(part 1 of 3)
# Autodesk Inventor assembly: COMPONENTS
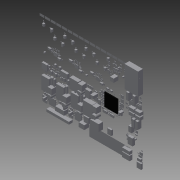
[picture p0: Inventor's stored thumbnail of the model, 180x180]
Saved by Autodesk Inventor 2016 (Build 200138000, 138)
## iProperties
Created: 2016-03-07
Part Number: COMPONENTS
Document SubType Name: Assembly
Designer: rtreacy
Author: rtreacy
## Documents named in this file (794)
- C:\Users\Dave\Desktop\hera-cad\SNAP\components\COMPONENTS.iam
- C:\Users\Dave\Desktop\hera-cad\SNAP\components\INDC1005X55L_L30.ipt
- C:\Users\Dave\Desktop\hera-cad\SNAP\components\INDC1005X55L_L31.ipt
- C:\Users\Dave\Desktop\hera-cad\SNAP\NRAO-LOGO_NOREFDES.ipt
- C:\Users\Dave\Desktop\hera-cad\SNAP\components\MOLEX_SD-74754-0220_M23.ipt
- C:\Users\Dave\Desktop\hera-cad\SNAP\SHDRRA14W55P200_7X2_1665X100-1_J11.ipt
- C:\Users\Dave\Desktop\hera-cad\SNAP\SHDRV14W55P200_7X2_1665X630H-1_J3.ipt
- C:\Users\Dave\Desktop\hera-cad\SNAP\components\TE_CONN_6367550-5_P3.ipt
- C:\Users\Dave\Desktop\hera-cad\SNAP\TO170P1430X470-6N-ALT1_U18.ipt
- C:\Users\Dave\Desktop\hera-cad\SNAP\components\SMA_END_LAUNCH_SMATP1.ipt
- C:\Users\Dave\Desktop\hera-cad\SNAP\components\SMA_END_LAUNCH_SMATP2.ipt
- C:\Users\Dave\Desktop\hera-cad\SNAP\components\SMA_END_LAUNCH_SMATP3.ipt
- C:\Users\Dave\Desktop\hera-cad\SNAP\components\SMA_END_LAUNCH_SMATP4.ipt
- C:\Users\Dave\Desktop\hera-cad\SNAP\components\SMA_END_LAUNCH_SMATP5.ipt
- C:\Users\Dave\Desktop\hera-cad\SNAP\components\SMA_END_LAUNCH_SMATP6.ipt
- C:\Users\Dave\Desktop\hera-cad\SNAP\components\SMA_END_LAUNCH_SMATP7.ipt
- C:\Users\Dave\Desktop\hera-cad\SNAP\components\SMA_END_LAUNCH_SMATP8.ipt
- C:\Users\Dave\Desktop\hera-cad\SNAP\components\SMA_END_LAUNCH_SMATP9.ipt
- C:\Users\Dave\Desktop\hera-cad\SNAP\components\SMA_END_LAUNCH_SMATP10.ipt
- C:\Users\Dave\Desktop\hera-cad\SNAP\components\SMA_END_LAUNCH_SMATP11.ipt
- C:\Users\Dave\Desktop\hera-cad\SNAP\components\SMA_END_LAUNCH_SMATP12.ipt
- C:\Users\Dave\Desktop\hera-cad\SNAP\components\SMA_END_LAUNCH_SMATP13.ipt
- C:\Users\Dave\Desktop\hera-cad\SNAP\components\SMA_END_LAUNCH_SMATP14.ipt
- C:\Users\Dave\Desktop\hera-cad\SNAP\components\SMA_END_LAUNCH_SMATP15.ipt
- C:\Users\Dave\Desktop\hera-cad\SNAP\components\SMA_END_LAUNCH_SMATP16.ipt
- C:\Users\Dave\Desktop\hera-cad\SNAP\components\HDRV254W64P254R1L508T254H838_JP3.ipt
- C:\Users\Dave\Desktop\hera-cad\SNAP\components\HDRV254W64P254R1L508T254H838_JP2.ipt
- C:\Users\Dave\Desktop\hera-cad\SNAP\components\HDRV254W64P254R1L508T254H838_JP1.ipt
- C:\Users\Dave\Desktop\hera-cad\SNAP\components\HDRV254W64P254R1L508T254H838_JP4.ipt
- C:\Users\Dave\Desktop\hera-cad\SNAP\components\HDRV6X2_J9.ipt
- C:\Users\Dave\Desktop\hera-cad\SNAP\components\HDRV6X2_J7.ipt
- C:\Users\Dave\Desktop\hera-cad\SNAP\components\HDRV6X2_J5.ipt
- C:\Users\Dave\Desktop\hera-cad\SNAP\components\HDRV6X2_J6.ipt
- C:\Users\Dave\Desktop\hera-cad\SNAP\components\HDRV2X20_PI2.ipt
- C:\Users\Dave\Desktop\hera-cad\SNAP\components\CAPPRD350W60D820H1170P_C259.ipt
- C:\Users\Dave\Desktop\hera-cad\SNAP\components\CAPPRD350W60D820H1170P_C250.ipt
- C:\Users\Dave\Desktop\hera-cad\SNAP\components\CAPPRD350W60D820H1170P_C241.ipt
- C:\Users\Dave\Desktop\hera-cad\SNAP\components\CAPPRD350W60D820H1170P_C234.ipt
- C:\Users\Dave\Desktop\hera-cad\SNAP\components\CAPPRD350W60D820H1170P_C227.ipt
- C:\Users\Dave\Desktop\hera-cad\SNAP\components\QFN50P500X500X100-28N_U29.ipt
- C:\Users\Dave\Desktop\hera-cad\SNAP\components\FID100X125_NOREFDES.ipt
- C:\Users\Dave\Desktop\hera-cad\SNAP\components\DIOAD1365W102L865D350B_D4.ipt
- C:\Users\Dave\Desktop\hera-cad\SNAP\components\DIOAD1365W102L865D350B_D5.ipt
- C:\Users\Dave\Desktop\hera-cad\SNAP\components\DIOAD1365W102L865D350B_D6.ipt
- C:\Users\Dave\Desktop\hera-cad\SNAP\components\DIOAD1365W102L865D350B_D7.ipt
- C:\Users\Dave\Desktop\hera-cad\SNAP\components\DIOAD1365W102L865D350B_D8.ipt
- C:\Users\Dave\Desktop\hera-cad\SNAP\BGA676C100P26X26_2700X2700X260_U25.ipt
- C:\Users\Dave\Desktop\hera-cad\SNAP\components\EMERSON_RFCONN_SMA-V_TP2.ipt
- C:\Users\Dave\Desktop\hera-cad\SNAP\components\FIL_BNX01X_U24.ipt
- C:\Users\Dave\Desktop\hera-cad\SNAP\components\MOLEX_744410010_P2.ipt
- C:\Users\Dave\Desktop\hera-cad\SNAP\components\MOLEX_744410010_P1.ipt
- C:\Users\Dave\Desktop\hera-cad\SNAP\components\SOT89_Q5.ipt
- C:\Users\Dave\Desktop\hera-cad\SNAP\components\SOT89_Q6.ipt
- C:\Users\Dave\Desktop\hera-cad\SNAP\components\QFN80P1000X1000X440-42T320X130X2N-ALT1_U20.ipt
- C:\Users\Dave\Desktop\hera-cad\SNAP\components\HDR_1X2_LOCK_MOLEX_J61.ipt
- C:\Users\Dave\Desktop\hera-cad\SNAP\components\DIOMELF3514_D14.ipt
- C:\Users\Dave\Desktop\hera-cad\SNAP\components\SOT230P700X180-4L050N_Q17.ipt
- C:\Users\Dave\Desktop\hera-cad\SNAP\components\QFP50P1400X1400X100-80N_U40.ipt
- C:\Users\Dave\Desktop\hera-cad\SNAP\components\QFP50P1400X1400X100-80N_U42.ipt
- C:\Users\Dave\Desktop\hera-cad\SNAP\components\QFN50P700X700X100-49T540X540L_U7.ipt
- C:\Users\Dave\Desktop\hera-cad\SNAP\components\QFN50P700X700X100-49T540X540L_U2.ipt
- C:\Users\Dave\Desktop\hera-cad\SNAP\components\QFN50P700X700X100-49T540X540L_U12.ipt
- C:\Users\Dave\Desktop\hera-cad\SNAP\components\QFN50P500X500X100-33T320X320L_U21.ipt
- C:\Users\Dave\Desktop\hera-cad\SNAP\components\QFN50P500X500X100-33T380X380L_U23.ipt
- C:\Users\Dave\Desktop\hera-cad\SNAP\components\QFN50P400X400X100-25T280X280L_U22.ipt
- C:\Users\Dave\Desktop\hera-cad\SNAP\components\DCDC-CONV_PTD08D210W-22N_U38.ipt
- C:\Users\Dave\Desktop\hera-cad\SNAP\components\DCDC-CONV_PTD08D210W-22N_U36.ipt
- C:\Users\Dave\Desktop\hera-cad\SNAP\components\DCDC-CONV_PTD08D210W-22N_U37.ipt
- C:\Users\Dave\Desktop\hera-cad\SNAP\components\QFN50P300X300X100-17T178X178L_U17.ipt
- C:\Users\Dave\Desktop\hera-cad\SNAP\components\QFN50P300X300X100-17T178X178L_U16.ipt
- C:\Users\Dave\Desktop\hera-cad\SNAP\components\SOP65P640X120-16N_U41.ipt
- C:\Users\Dave\Desktop\hera-cad\SNAP\components\SOP65P640X120-16N_U39.ipt
- C:\Users\Dave\Desktop\hera-cad\SNAP\components\QFN40P260X180X55-16L_U28.ipt
- C:\Users\Dave\Desktop\hera-cad\SNAP\components\QFN40P260X180X55-16L_U46.ipt
- C:\Users\Dave\Desktop\hera-cad\SNAP\components\QFN40P260X180X55-16L_U47.ipt
- C:\Users\Dave\Desktop\hera-cad\SNAP\components\DCDC-CONV_PTD08A020WAD-12N_U35.ipt
- C:\Users\Dave\Desktop\hera-cad\SNAP\components\DCDC-CONV_PTD08A010WAD-12N_U34.ipt
- C:\Users\Dave\Desktop\hera-cad\SNAP\components\HDRV1016W64P254R2L2032T905H900_J1.ipt
- C:\Users\Dave\Desktop\hera-cad\SNAP\components\SW_SDA05H1SBD_S2.ipt
- C:\Users\Dave\Desktop\hera-cad\SNAP\components\SW_SDA05H1SBD_S1.ipt
- C:\Users\Dave\Desktop\hera-cad\SNAP\components\MOLEX_548190589_J4.ipt
- C:\Users\Dave\Desktop\hera-cad\SNAP\components\SOP50P310X90-8N_U44.ipt
- C:\Users\Dave\Desktop\hera-cad\SNAP\components\SOP50P310X90-8N_U45.ipt
- C:\Users\Dave\Desktop\hera-cad\SNAP\components\OSC254P700X500X90-7T147X230N_U32.ipt
- C:\Users\Dave\Desktop\hera-cad\SNAP\components\MOLEX_39301060_J2.ipt
- C:\Users\Dave\Desktop\hera-cad\SNAP\components\SOT95P280X145-6N_U26.ipt
- C:\Users\Dave\Desktop\hera-cad\SNAP\components\OSC254P700X500X90-6N_U48.ipt
- C:\Users\Dave\Desktop\hera-cad\SNAP\components\OSC254P700X500X90-6N_U33.ipt
- C:\Users\Dave\Desktop\hera-cad\SNAP\components\XFMR_TC1-1-13MG2_T11.ipt
- C:\Users\Dave\Desktop\hera-cad\SNAP\components\XFMR_TC1-1-13MG2_T10.ipt
- C:\Users\Dave\Desktop\hera-cad\SNAP\components\XFMR_TC1-1-13MG2_T4.ipt
- C:\Users\Dave\Desktop\hera-cad\SNAP\components\XFMR_TC1-1-13MG2_T6.ipt
- C:\Users\Dave\Desktop\hera-cad\SNAP\components\XFMR_TC1-1-13MG2_T12.ipt
- C:\Users\Dave\Desktop\hera-cad\SNAP\components\XFMR_TC1-1-13MG2_T5.ipt
- C:\Users\Dave\Desktop\hera-cad\SNAP\components\XFMR_TC1-1-13MG2_T3.ipt
- C:\Users\Dave\Desktop\hera-cad\SNAP\components\XFMR_TC1-1-13MG2_T8.ipt
- C:\Users\Dave\Desktop\hera-cad\SNAP\components\XFMR_TC1-1-13MG2_T9.ipt
- C:\Users\Dave\Desktop\hera-cad\SNAP\components\XFMR_TC1-1-13MG2_T13.ipt
- C:\Users\Dave\Desktop\hera-cad\SNAP\components\XFMR_TC1-1-13MG2_T2.ipt
- C:\Users\Dave\Desktop\hera-cad\SNAP\components\XFMR_TC1-1-13MG2_T7.ipt
- C:\Users\Dave\Desktop\hera-cad\SNAP\components\XFMR_TC1-1-13MG2_T1.ipt
- C:\Users\Dave\Desktop\hera-cad\SNAP\components\SOT95P280X145-5N_U30.ipt
- C:\Users\Dave\Desktop\hera-cad\SNAP\components\SOT95P280X145-5N_U19.ipt
- C:\Users\Dave\Desktop\hera-cad\SNAP\components\SOT143R_X1.ipt
- C:\Users\Dave\Desktop\hera-cad\SNAP\components\RESCAF65P100X100X45-4N_U10.ipt
- C:\Users\Dave\Desktop\hera-cad\SNAP\components\RESCAF65P100X100X45-4N_U1.ipt
- C:\Users\Dave\Desktop\hera-cad\SNAP\components\RESCAF65P100X100X45-4N_U11.ipt
- C:\Users\Dave\Desktop\hera-cad\SNAP\components\RESCAF65P100X100X45-4N_U13.ipt
- C:\Users\Dave\Desktop\hera-cad\SNAP\components\RESCAF65P100X100X45-4N_U14.ipt
- C:\Users\Dave\Desktop\hera-cad\SNAP\components\RESCAF65P100X100X45-4N_U15.ipt
- C:\Users\Dave\Desktop\hera-cad\SNAP\components\RESCAF65P100X100X45-4N_U3.ipt
- C:\Users\Dave\Desktop\hera-cad\SNAP\components\RESCAF65P100X100X45-4N_U4.ipt
- C:\Users\Dave\Desktop\hera-cad\SNAP\components\RESCAF65P100X100X45-4N_U5.ipt
- C:\Users\Dave\Desktop\hera-cad\SNAP\components\RESCAF65P100X100X45-4N_U6.ipt
- C:\Users\Dave\Desktop\hera-cad\SNAP\components\RESCAF65P100X100X45-4N_U8.ipt
- C:\Users\Dave\Desktop\hera-cad\SNAP\components\RESCAF65P100X100X45-4N_U9.ipt
- C:\Users\Dave\Desktop\hera-cad\SNAP\components\SW_TL3301EF100QG_SW5.ipt
- C:\Users\Dave\Desktop\hera-cad\SNAP\components\SW_TL3301EF100QG_SW4.ipt
- C:\Users\Dave\Desktop\hera-cad\SNAP\components\SW_TL3301EF100QG_SW3.ipt
- C:\Users\Dave\Desktop\hera-cad\SNAP\components\SW_TL3301EF100QG_SW2.ipt
- C:\Users\Dave\Desktop\hera-cad\SNAP\components\SW_TL3301EF100QG_SW1.ipt
- C:\Users\Dave\Desktop\hera-cad\SNAP\components\SOT192P237X112-4L20N_D3.ipt
- C:\Users\Dave\Desktop\hera-cad\SNAP\components\SOT95P237X100-4_Q1.ipt
- C:\Users\Dave\Desktop\hera-cad\SNAP\components\SOT95P237X100-4_Q4.ipt
- C:\Users\Dave\Desktop\hera-cad\SNAP\components\SOT95P237X100-4_Q3.ipt
- C:\Users\Dave\Desktop\hera-cad\SNAP\components\SOT95P237X100-4_Q2.ipt
- C:\Users\Dave\Desktop\hera-cad\SNAP\components\SOT95P237X100-4_Q8.ipt
- C:\Users\Dave\Desktop\hera-cad\SNAP\components\SOT95P237X100-4_Q7.ipt
- C:\Users\Dave\Desktop\hera-cad\SNAP\components\SOT95P240X110-3L16N_U31.ipt
- C:\Users\Dave\Desktop\hera-cad\SNAP\components\SOT95P240X110-3L16N_D1.ipt
- C:\Users\Dave\Desktop\hera-cad\SNAP\components\SOT95P240X110-3L16N_D2.ipt
- C:\Users\Dave\Desktop\hera-cad\SNAP\components\CAPC1005X50L_C604.ipt
- C:\Users\Dave\Desktop\hera-cad\SNAP\components\CAPC1005X50L_C603.ipt
- C:\Users\Dave\Desktop\hera-cad\SNAP\components\CAPC1005X50L_C591.ipt
- C:\Users\Dave\Desktop\hera-cad\SNAP\components\CAPC1005X50L_C592.ipt
- C:\Users\Dave\Desktop\hera-cad\SNAP\components\CAPC1005X50L_C593.ipt
- C:\Users\Dave\Desktop\hera-cad\SNAP\components\CAPC1005X50L_C46.ipt
- C:\Users\Dave\Desktop\hera-cad\SNAP\components\CAPC1005X50L_C51.ipt
- C:\Users\Dave\Desktop\hera-cad\SNAP\components\CAPC1005X50L_C57.ipt
- C:\Users\Dave\Desktop\hera-cad\SNAP\components\CAPC1005X50L_C7.ipt
- C:\Users\Dave\Desktop\hera-cad\SNAP\components\CAPC1005X50L_C82.ipt
- C:\Users\Dave\Desktop\hera-cad\SNAP\components\CAPC1005X50L_C43.ipt
- C:\Users\Dave\Desktop\hera-cad\SNAP\components\CAPC1005X50L_C96.ipt
- C:\Users\Dave\Desktop\hera-cad\SNAP\components\CAPC1005X50L_C85.ipt
- C:\Users\Dave\Desktop\hera-cad\SNAP\components\CAPC1005X50L_C90.ipt
- C:\Users\Dave\Desktop\hera-cad\SNAP\components\CAPC1005X50L_C13.ipt
- C:\Users\Dave\Desktop\hera-cad\SNAP\components\CAPC1005X50L_C4.ipt
- C:\Users\Dave\Desktop\hera-cad\SNAP\components\CAPC1005X50L_C47.ipt
- C:\Users\Dave\Desktop\hera-cad\SNAP\components\CAPC1005X50L_C5.ipt
- C:\Users\Dave\Desktop\hera-cad\SNAP\components\CAPC1005X50L_C52.ipt
- C:\Users\Dave\Desktop\hera-cad\SNAP\components\CAPC1005X50L_C58.ipt
- C:\Users\Dave\Desktop\hera-cad\SNAP\components\CAPC1005X50L_C8.ipt
- C:\Users\Dave\Desktop\hera-cad\SNAP\components\CAPC1005X50L_C83.ipt
- C:\Users\Dave\Desktop\hera-cad\SNAP\components\CAPC1005X50L_C86.ipt
- C:\Users\Dave\Desktop\hera-cad\SNAP\components\CAPC1005X50L_C91.ipt
- C:\Users\Dave\Desktop\hera-cad\SNAP\components\CAPC1005X50L_C97.ipt
- C:\Users\Dave\Desktop\hera-cad\SNAP\components\CAPC1005X50L_C19.ipt
- C:\Users\Dave\Desktop\hera-cad\SNAP\components\CAPC1005X50L_C14.ipt
- C:\Users\Dave\Desktop\hera-cad\SNAP\components\CAPC1005X50L_C17.ipt
- C:\Users\Dave\Desktop\hera-cad\SNAP\components\CAPC1005X50L_C2.ipt
- C:\Users\Dave\Desktop\hera-cad\SNAP\components\CAPC1005X50L_C41.ipt
- C:\Users\Dave\Desktop\hera-cad\SNAP\components\CAPC1005X50L_C44.ipt
- C:\Users\Dave\Desktop\hera-cad\SNAP\components\CAPC1005X50L_C53.ipt
- C:\Users\Dave\Desktop\hera-cad\SNAP\components\CAPC1005X50L_C80.ipt
- C:\Users\Dave\Desktop\hera-cad\SNAP\components\CAPC1005X50L_C87.ipt
- C:\Users\Dave\Desktop\hera-cad\SNAP\components\CAPC1005X50L_C9.ipt
- C:\Users\Dave\Desktop\hera-cad\SNAP\components\CAPC1005X50L_C92.ipt
- C:\Users\Dave\Desktop\hera-cad\SNAP\components\CAPC1005X50L_C95.ipt
- C:\Users\Dave\Desktop\hera-cad\SNAP\components\CAPC1005X50L_C48.ipt
- C:\Users\Dave\Desktop\hera-cad\SNAP\components\CAPC1005X50L_C148.ipt
- C:\Users\Dave\Desktop\hera-cad\SNAP\components\CAPC1005X50L_C56.ipt
- C:\Users\Dave\Desktop\hera-cad\SNAP\components\CAPC1005X50L_C194.ipt
- C:\Users\Dave\Desktop\hera-cad\SNAP\components\CAPC1005X50L_C195.ipt
- C:\Users\Dave\Desktop\hera-cad\SNAP\components\CAPC1005X50L_C217.ipt
- C:\Users\Dave\Desktop\hera-cad\SNAP\components\CAPC1005X50L_C219.ipt
- C:\Users\Dave\Desktop\hera-cad\SNAP\components\CAPC1005X50L_C220.ipt
- C:\Users\Dave\Desktop\hera-cad\SNAP\components\CAPC1005X50L_C222.ipt
- C:\Users\Dave\Desktop\hera-cad\SNAP\components\CAPC1005X50L_C223.ipt
- C:\Users\Dave\Desktop\hera-cad\SNAP\components\CAPC1005X50L_C224.ipt
- C:\Users\Dave\Desktop\hera-cad\SNAP\components\CAPC1005X50L_C225.ipt
- C:\Users\Dave\Desktop\hera-cad\SNAP\components\CAPC1005X50L_C226.ipt
- C:\Users\Dave\Desktop\hera-cad\SNAP\components\CAPC1005X50L_C269.ipt
- C:\Users\Dave\Desktop\hera-cad\SNAP\components\CAPC1005X50L_C270.ipt
- C:\Users\Dave\Desktop\hera-cad\SNAP\components\CAPC1005X50L_C271.ipt
- C:\Users\Dave\Desktop\hera-cad\SNAP\components\CAPC1005X50L_C273.ipt
- C:\Users\Dave\Desktop\hera-cad\SNAP\components\CAPC1005X50L_C275.ipt
- C:\Users\Dave\Desktop\hera-cad\SNAP\components\CAPC1005X50L_C276.ipt
- C:\Users\Dave\Desktop\hera-cad\SNAP\components\CAPC1005X50L_C277.ipt
- C:\Users\Dave\Desktop\hera-cad\SNAP\components\CAPC1005X50L_C285.ipt
- C:\Users\Dave\Desktop\hera-cad\SNAP\components\CAPC1005X50L_C286.ipt
- C:\Users\Dave\Desktop\hera-cad\SNAP\components\CAPC1005X50L_C291.ipt
- C:\Users\Dave\Desktop\hera-cad\SNAP\components\CAPC1005X50L_C292.ipt
- C:\Users\Dave\Desktop\hera-cad\SNAP\components\CAPC1005X50L_C293.ipt
- C:\Users\Dave\Desktop\hera-cad\SNAP\components\CAPC1005X50L_C295.ipt
- C:\Users\Dave\Desktop\hera-cad\SNAP\components\CAPC1005X50L_C297.ipt
- C:\Users\Dave\Desktop\hera-cad\SNAP\components\CAPC1005X50L_C298.ipt
- C:\Users\Dave\Desktop\hera-cad\SNAP\components\CAPC1005X50L_C299.ipt
- C:\Users\Dave\Desktop\hera-cad\SNAP\components\CAPC1005X50L_C307.ipt
- C:\Users\Dave\Desktop\hera-cad\SNAP\components\CAPC1005X50L_C308.ipt
- C:\Users\Dave\Desktop\hera-cad\SNAP\components\CAPC1005X50L_C312.ipt
- C:\Users\Dave\Desktop\hera-cad\SNAP\components\CAPC1005X50L_C313.ipt
- C:\Users\Dave\Desktop\hera-cad\SNAP\components\CAPC1005X50L_C315.ipt
- C:\Users\Dave\Desktop\hera-cad\SNAP\components\CAPC1005X50L_C317.ipt
- C:\Users\Dave\Desktop\hera-cad\SNAP\components\CAPC1005X50L_C318.ipt
- C:\Users\Dave\Desktop\hera-cad\SNAP\components\CAPC1005X50L_C319.ipt
- C:\Users\Dave\Desktop\hera-cad\SNAP\components\CAPC1005X50L_C321.ipt
- C:\Users\Dave\Desktop\hera-cad\SNAP\components\CAPC1005X50L_C323.ipt
- C:\Users\Dave\Desktop\hera-cad\SNAP\components\CAPC1005X50L_C324.ipt
- C:\Users\Dave\Desktop\hera-cad\SNAP\components\CAPC1005X50L_C325.ipt
- C:\Users\Dave\Desktop\hera-cad\SNAP\components\CAPC1005X50L_C326.ipt
- C:\Users\Dave\Desktop\hera-cad\SNAP\components\CAPC1005X50L_C327.ipt
- C:\Users\Dave\Desktop\hera-cad\SNAP\components\CAPC1005X50L_C328.ipt
- C:\Users\Dave\Desktop\hera-cad\SNAP\components\CAPC1005X50L_C15.ipt
- C:\Users\Dave\Desktop\hera-cad\SNAP\components\CAPC1005X50L_C54.ipt
- C:\Users\Dave\Desktop\hera-cad\SNAP\components\CAPC1005X50L_C192.ipt
- C:\Users\Dave\Desktop\hera-cad\SNAP\components\CAPC1005X50L_C151.ipt
- C:\Users\Dave\Desktop\hera-cad\SNAP\components\CAPC1005X50L_C152.ipt
- C:\Users\Dave\Desktop\hera-cad\SNAP\components\CAPC1005X50L_C153.ipt
- C:\Users\Dave\Desktop\hera-cad\SNAP\components\CAPC1005X50L_C154.ipt
- C:\Users\Dave\Desktop\hera-cad\SNAP\components\CAPC1005X50L_C157.ipt
- C:\Users\Dave\Desktop\hera-cad\SNAP\components\CAPC1005X50L_C160.ipt
- C:\Users\Dave\Desktop\hera-cad\SNAP\components\CAPC1005X50L_C164.ipt
- C:\Users\Dave\Desktop\hera-cad\SNAP\components\CAPC1005X50L_C167.ipt
- C:\Users\Dave\Desktop\hera-cad\SNAP\components\CAPC1005X50L_C172.ipt
- C:\Users\Dave\Desktop\hera-cad\SNAP\components\CAPC1005X50L_C176.ipt
- C:\Users\Dave\Desktop\hera-cad\SNAP\components\CAPC1005X50L_C178.ipt
- C:\Users\Dave\Desktop\hera-cad\SNAP\components\CAPC1005X50L_C16.ipt
- C:\Users\Dave\Desktop\hera-cad\SNAP\components\CAPC1005X50L_C55.ipt
- C:\Users\Dave\Desktop\hera-cad\SNAP\components\CAPC1005X50L_C94.ipt
- C:\Users\Dave\Desktop\hera-cad\SNAP\components\CAPC1005X50L_C168.ipt
- C:\Users\Dave\Desktop\hera-cad\SNAP\components\CAPC1005X50L_C173.ipt
- C:\Users\Dave\Desktop\hera-cad\SNAP\components\CAPC1005X50L_C177.ipt
- C:\Users\Dave\Desktop\hera-cad\SNAP\components\CAPC1005X50L_C180.ipt
- C:\Users\Dave\Desktop\hera-cad\SNAP\components\CAPC1005X50L_C216.ipt
- C:\Users\Dave\Desktop\hera-cad\SNAP\components\CAPC1005X50L_C184.ipt
- C:\Users\Dave\Desktop\hera-cad\SNAP\components\CAPC1005X50L_C187.ipt
- C:\Users\Dave\Desktop\hera-cad\SNAP\components\CAPC1005X50L_C188.ipt
- C:\Users\Dave\Desktop\hera-cad\SNAP\components\CAPC1005X50L_C189.ipt
- C:\Users\Dave\Desktop\hera-cad\SNAP\components\CAPC1005X50L_C182.ipt
- C:\Users\Dave\Desktop\hera-cad\SNAP\components\CAPC1005X50L_C18.ipt
- C:\Users\Dave\Desktop\hera-cad\SNAP\components\CAPC1005X50L_C93.ipt
- C:\Users\Dave\Desktop\hera-cad\SNAP\components\CAPC1005X50L_C186.ipt
- C:\Users\Dave\Desktop\hera-cad\SNAP\components\CAPC1005X50L_C20.ipt
- C:\Users\Dave\Desktop\hera-cad\SNAP\components\CAPC1005X50L_C59.ipt
- C:\Users\Dave\Desktop\hera-cad\SNAP\components\CAPC1005X50L_C98.ipt
- C:\Users\Dave\Desktop\hera-cad\SNAP\components\CAPC1005X50L_C279.ipt
- C:\Users\Dave\Desktop\hera-cad\SNAP\components\CAPC1005X50L_C280.ipt
- C:\Users\Dave\Desktop\hera-cad\SNAP\components\CAPC1005X50L_C282.ipt
- C:\Users\Dave\Desktop\hera-cad\SNAP\components\CAPC1005X50L_C284.ipt
- C:\Users\Dave\Desktop\hera-cad\SNAP\components\CAPC1005X50L_C289.ipt
- C:\Users\Dave\Desktop\hera-cad\SNAP\components\CAPC1005X50L_C301.ipt
- C:\Users\Dave\Desktop\hera-cad\SNAP\components\CAPC1005X50L_C302.ipt
- C:\Users\Dave\Desktop\hera-cad\SNAP\components\CAPC1005X50L_C304.ipt
- C:\Users\Dave\Desktop\hera-cad\SNAP\components\CAPC1005X50L_C306.ipt
- C:\Users\Dave\Desktop\hera-cad\SNAP\components\CAPC1005X50L_C311.ipt
- C:\Users\Dave\Desktop\hera-cad\SNAP\components\CAPC1005X50L_C287.ipt
- C:\Users\Dave\Desktop\hera-cad\SNAP\components\CAPC1005X50L_C309.ipt
- C:\Users\Dave\Desktop\hera-cad\SNAP\components\CAPC1005X50L_C3.ipt
- C:\Users\Dave\Desktop\hera-cad\SNAP\components\CAPC1005X50L_C42.ipt
- C:\Users\Dave\Desktop\hera-cad\SNAP\components\CAPC1005X50L_C81.ipt
- C:\Users\Dave\Desktop\hera-cad\SNAP\components\CAPC1005X50L_C45.ipt
- C:\Users\Dave\Desktop\hera-cad\SNAP\components\CAPC1005X50L_C6.ipt
- C:\Users\Dave\Desktop\hera-cad\SNAP\components\CAPC1005X50L_C84.ipt
- C:\Users\Dave\Desktop\hera-cad\SNAP\components\CAPC1005X50L_C12.ipt
- C:\Users\Dave\Desktop\hera-cad\SNAP\components\CAPC1005X50L_C181.ipt
- C:\Users\Dave\Desktop\hera-cad\SNAP\components\CAPC1005X50L_C139.ipt
- C:\Users\Dave\Desktop\hera-cad\SNAP\components\CAPC1005X50L_C76.ipt
- C:\Users\Dave\Desktop\hera-cad\SNAP\components\CAPC1005X50L_C37.ipt
- C:\Users\Dave\Desktop\hera-cad\SNAP\components\CAPC1005X50L_C115.ipt
- C:\Users\Dave\Desktop\hera-cad\SNAP\components\CAPC1005X50L_C75.ipt
- C:\Users\Dave\Desktop\hera-cad\SNAP\components\CAPC1005X50L_C36.ipt
- C:\Users\Dave\Desktop\hera-cad\SNAP\components\CAPC1005X50L_C114.ipt
- C:\Users\Dave\Desktop\hera-cad\SNAP\components\CAPC1005X50L_C74.ipt
- C:\Users\Dave\Desktop\hera-cad\SNAP\components\CAPC1005X50L_C136.ipt
- C:\Users\Dave\Desktop\hera-cad\SNAP\components\CAPC1005X50L_C183.ipt
- C:\Users\Dave\Desktop\hera-cad\SNAP\components\CAPC1005X50L_C35.ipt
- C:\Users\Dave\Desktop\hera-cad\SNAP\components\CAPC1005X50L_C113.ipt
- C:\Users\Dave\Desktop\hera-cad\SNAP\components\CAPC1005X50L_C175.ipt
- C:\Users\Dave\Desktop\hera-cad\SNAP\components\CAPC1005X50L_C174.ipt
- C:\Users\Dave\Desktop\hera-cad\SNAP\components\CAPC1005X50L_C171.ipt
- C:\Users\Dave\Desktop\hera-cad\SNAP\components\CAPC1005X50L_C166.ipt
- C:\Users\Dave\Desktop\hera-cad\SNAP\components\CAPC1005X50L_C165.ipt
- C:\Users\Dave\Desktop\hera-cad\SNAP\components\CAPC1005X50L_C185.ipt
- C:\Users\Dave\Desktop\hera-cad\SNAP\components\CAPC1005X50L_C163.ipt
- C:\Users\Dave\Desktop\hera-cad\SNAP\components\CAPC1005X50L_C72.ipt
- C:\Users\Dave\Desktop\hera-cad\SNAP\components\CAPC1005X50L_C135.ipt
- C:\Users\Dave\Desktop\hera-cad\SNAP\components\CAPC1005X50L_C131.ipt
- C:\Users\Dave\Desktop\hera-cad\SNAP\components\CAPC1005X50L_C129.ipt
- C:\Users\Dave\Desktop\hera-cad\SNAP\components\CAPC1005X50L_C127.ipt
- C:\Users\Dave\Desktop\hera-cad\SNAP\components\CAPC1005X50L_C123.ipt
- C:\Users\Dave\Desktop\hera-cad\SNAP\components\CAPC1005X50L_C33.ipt
- C:\Users\Dave\Desktop\hera-cad\SNAP\components\CAPC1005X50L_C111.ipt
- C:\Users\Dave\Desktop\hera-cad\SNAP\components\CAPC1005X50L_C89.ipt
- C:\Users\Dave\Desktop\hera-cad\SNAP\components\CAPC1005X50L_C50.ipt
- C:\Users\Dave\Desktop\hera-cad\SNAP\components\CAPC1005X50L_C11.ipt
- C:\Users\Dave\Desktop\hera-cad\SNAP\components\CAPC1005X50L_C70.ipt
- C:\Users\Dave\Desktop\hera-cad\SNAP\components\CAPC1005X50L_C31.ipt
- C:\Users\Dave\Desktop\hera-cad\SNAP\components\CAPC1005X50L_C109.ipt
- C:\Users\Dave\Desktop\hera-cad\SNAP\components\CAPC1005X50L_C69.ipt
- C:\Users\Dave\Desktop\hera-cad\SNAP\components\CAPC1005X50L_C30.ipt
- C:\Users\Dave\Desktop\hera-cad\SNAP\components\CAPC1005X50L_C121.ipt
- C:\Users\Dave\Desktop\hera-cad\SNAP\components\CAPC1005X50L_C119.ipt
- C:\Users\Dave\Desktop\hera-cad\SNAP\components\CAPC1005X50L_C108.ipt
- C:\Users\Dave\Desktop\hera-cad\SNAP\components\CAPC1005X50L_C78.ipt
- C:\Users\Dave\Desktop\hera-cad\SNAP\components\CAPC1005X50L_C39.ipt
- C:\Users\Dave\Desktop\hera-cad\SNAP\components\CAPC1005X50L_C117.ipt
- C:\Users\Dave\Desktop\hera-cad\SNAP\components\CAPC1005X50L_C104.ipt
- C:\Users\Dave\Desktop\hera-cad\SNAP\components\CAPC1005X50L_C64.ipt
- C:\Users\Dave\Desktop\hera-cad\SNAP\components\CAPC1005X50L_C1.ipt
- C:\Users\Dave\Desktop\hera-cad\SNAP\components\CAPC1005X50L_C40.ipt
- C:\Users\Dave\Desktop\hera-cad\SNAP\components\CAPC1005X50L_C79.ipt
- C:\Users\Dave\Desktop\hera-cad\SNAP\components\CAPC1005X50L_C10.ipt
- C:\Users\Dave\Desktop\hera-cad\SNAP\components\CAPC1005X50L_C49.ipt
- C:\Users\Dave\Desktop\hera-cad\SNAP\components\CAPC1005X50L_C88.ipt
- C:\Users\Dave\Desktop\hera-cad\SNAP\components\CAPC1005X50L_C67.ipt
- C:\Users\Dave\Desktop\hera-cad\SNAP\components\CAPC1005X50L_C28.ipt
- C:\Users\Dave\Desktop\hera-cad\SNAP\components\CAPC1005X50L_C106.ipt
- C:\Users\Dave\Desktop\hera-cad\SNAP\components\CAPC1005X50L_C66.ipt
- C:\Users\Dave\Desktop\hera-cad\SNAP\components\CAPC1005X50L_C27.ipt
- C:\Users\Dave\Desktop\hera-cad\SNAP\components\CAPC1005X50L_C105.ipt
- C:\Users\Dave\Desktop\hera-cad\SNAP\components\CAPC1005X50L_C65.ipt
- C:\Users\Dave\Desktop\hera-cad\SNAP\components\CAPC1005X50L_C26.ipt
- C:\Users\Dave\Desktop\hera-cad\SNAP\components\CAPC1005X50L_C25.ipt
- C:\Users\Dave\Desktop\hera-cad\SNAP\components\CAPC1005X50L_C102.ipt
- C:\Users\Dave\Desktop\hera-cad\SNAP\components\CAPC1005X50L_C103.ipt
- C:\Users\Dave\Desktop\hera-cad\SNAP\components\CAPC1005X50L_C63.ipt
- C:\Users\Dave\Desktop\hera-cad\SNAP\components\CAPC1005X50L_C24.ipt
- C:\Users\Dave\Desktop\hera-cad\SNAP\components\CAPC1005X50L_C61.ipt
- C:\Users\Dave\Desktop\hera-cad\SNAP\components\CAPC1005X50L_C100.ipt
- C:\Users\Dave\Desktop\hera-cad\SNAP\components\CAPC1005X50L_C22.ipt
- C:\Users\Dave\Desktop\hera-cad\SNAP\components\CAPC1005X50L_C601.ipt
- C:\Users\Dave\Desktop\hera-cad\SNAP\components\CAPC1005X50L_C602.ipt
- C:\Users\Dave\Desktop\hera-cad\SNAP\components\CAPC1608X90N_C120.ipt
- C:\Users\Dave\Desktop\hera-cad\SNAP\components\CAPC1608X90N_C124.ipt
- C:\Users\Dave\Desktop\hera-cad\SNAP\components\CAPC1608X90N_C128.ipt
- C:\Users\Dave\Desktop\hera-cad\SNAP\components\CAPC1608X90N_C132.ipt
- C:\Users\Dave\Desktop\hera-cad\SNAP\components\CAPC1608X90N_C179.ipt
- C:\Users\Dave\Desktop\hera-cad\SNAP\components\CAPC1608X90N_C150.ipt
- C:\Users\Dave\Desktop\hera-cad\SNAP\components\CAPC1608X90N_C140.ipt
- C:\Users\Dave\Desktop\hera-cad\SNAP\components\CAPC1608X90N_C161.ipt
- C:\Users\Dave\Desktop\hera-cad\SNAP\components\CAPC1608X90N_C169.ipt
- C:\Users\Dave\Desktop\hera-cad\SNAP\components\CAPC1608X90N_C190.ipt
- C:\Users\Dave\Desktop\hera-cad\SNAP\components\CAPC1608X90N_C218.ipt
- C:\Users\Dave\Desktop\hera-cad\SNAP\components\CAPC1608X90N_C221.ipt
- C:\Users\Dave\Desktop\hera-cad\SNAP\components\CAPC1608X90N_C229.ipt
- C:\Users\Dave\Desktop\hera-cad\SNAP\components\CAPC1608X90N_C236.ipt
- C:\Users\Dave\Desktop\hera-cad\SNAP\components\CAPC1608X90N_C243.ipt
- C:\Users\Dave\Desktop\hera-cad\SNAP\components\CAPC1608X90N_C252.ipt
- C:\Users\Dave\Desktop\hera-cad\SNAP\components\CAPC1608X90N_C261.ipt
- C:\Users\Dave\Desktop\hera-cad\SNAP\components\CAPC1608X90N_C193.ipt
- C:\Users\Dave\Desktop\hera-cad\SNAP\components\CAPC1608X90N_C215.ipt
- C:\Users\Dave\Desktop\hera-cad\SNAP\components\CAPC1608X90N_C21.ipt
- C:\Users\Dave\Desktop\hera-cad\SNAP\components\CAPC1608X90N_C60.ipt
- C:\Users\Dave\Desktop\hera-cad\SNAP\components\CAPC1608X90N_C99.ipt
- C:\Users\Dave\Desktop\hera-cad\SNAP\components\CAPC1608X90N_C38.ipt
- C:\Users\Dave\Desktop\hera-cad\SNAP\components\CAPC1608X90N_C116.ipt
- C:\Users\Dave\Desktop\hera-cad\SNAP\components\CAPC1608X90N_C73.ipt
- C:\Users\Dave\Desktop\hera-cad\SNAP\components\CAPC1608X90N_C34.ipt
- C:\Users\Dave\Desktop\hera-cad\SNAP\components\CAPC1608X90N_C112.ipt
- C:\Users\Dave\Desktop\hera-cad\SNAP\components\CAPC1608X90N_C71.ipt
- C:\Users\Dave\Desktop\hera-cad\SNAP\components\CAPC1608X90N_C32.ipt
- C:\Users\Dave\Desktop\hera-cad\SNAP\components\CAPC1608X90N_C110.ipt
- C:\Users\Dave\Desktop\hera-cad\SNAP\components\CAPC1608X90N_C77.ipt
- C:\Users\Dave\Desktop\hera-cad\SNAP\components\CAPC1608X90N_C68.ipt
- C:\Users\Dave\Desktop\hera-cad\SNAP\components\CAPC1608X90N_C29.ipt
- C:\Users\Dave\Desktop\hera-cad\SNAP\components\CAPC1608X90N_C107.ipt
- C:\Users\Dave\Desktop\hera-cad\SNAP\components\CAPC1608X90N_C62.ipt
- C:\Users\Dave\Desktop\hera-cad\SNAP\components\CAPC1608X90N_C23.ipt
- C:\Users\Dave\Desktop\hera-cad\SNAP\components\CAPC1608X90N_C101.ipt
- C:\Users\Dave\Desktop\hera-cad\SNAP\components\CAPC3216X180N_C134.ipt
- C:\Users\Dave\Desktop\hera-cad\SNAP\components\CAPC3216X180N_C138.ipt
- C:\Users\Dave\Desktop\hera-cad\SNAP\components\CAPC3216X180N_C141.ipt
- C:\Users\Dave\Desktop\hera-cad\SNAP\components\CAPC3216X180N_C143.ipt
- C:\Users\Dave\Desktop\hera-cad\SNAP\components\CAPC3216X180N_C144.ipt
- C:\Users\Dave\Desktop\hera-cad\SNAP\components\CAPC3216X180N_C231.ipt
- C:\Users\Dave\Desktop\hera-cad\SNAP\components\CAPC3216X180N_C238.ipt
- C:\Users\Dave\Desktop\hera-cad\SNAP\components\CAPC3216X180N_C245.ipt
- C:\Users\Dave\Desktop\hera-cad\SNAP\components\CAPC3216X180N_C254.ipt
- C:\Users\Dave\Desktop\hera-cad\SNAP\components\CAPC3216X180N_C263.ipt
- C:\Users\Dave\Desktop\hera-cad\SNAP\components\CAPC3216X180N_C314.ipt
- C:\Users\Dave\Desktop\hera-cad\SNAP\components\CAPC3216X180N_C316.ipt
- C:\Users\Dave\Desktop\hera-cad\SNAP\components\CAPC3216X180N_C320.ipt
- C:\Users\Dave\Desktop\hera-cad\SNAP\components\CAPC3216X180N_C322.ipt
- C:\Users\Dave\Desktop\hera-cad\SNAP\components\CAPC3216X180N_C146.ipt
- C:\Users\Dave\Desktop\hera-cad\SNAP\components\CAPC3216X180N_C197.ipt
- C:\Users\Dave\Desktop\hera-cad\SNAP\components\CAPC3216X180N_C145.ipt
- C:\Users\Dave\Desktop\hera-cad\SNAP\components\CAPC3216X180N_C149.ipt
- C:\Users\Dave\Desktop\hera-cad\SNAP\components\CAPC3216X180N_C155.ipt
- C:\Users\Dave\Desktop\hera-cad\SNAP\components\CAPC3216X180N_C158.ipt
- C:\Users\Dave\Desktop\hera-cad\SNAP\components\CAPC3216X180N_C156.ipt
- C:\Users\Dave\Desktop\hera-cad\SNAP\components\CAPC3216X180N_C159.ipt
- C:\Users\Dave\Desktop\hera-cad\SNAP\components\CAPC3216X180N_C212.ipt
- C:\Users\Dave\Desktop\hera-cad\SNAP\components\CAPC3216X180N_C213.ipt
- C:\Users\Dave\Desktop\hera-cad\SNAP\components\CAPC3216X180N_C214.ipt
- C:\Users\Dave\Desktop\hera-cad\SNAP\components\CAPC3216X180N_C228.ipt
- C:\Users\Dave\Desktop\hera-cad\SNAP\components\CAPC3216X180N_C235.ipt
- C:\Users\Dave\Desktop\hera-cad\SNAP\components\CAPC3216X180N_C242.ipt
- C:\Users\Dave\Desktop\hera-cad\SNAP\components\CAPC3216X180N_C251.ipt
- C:\Users\Dave\Desktop\hera-cad\SNAP\components\CAPC3216X180N_C260.ipt
- C:\Users\Dave\Desktop\hera-cad\SNAP\components\CAPC3216X180N_C232.ipt
- C:\Users\Dave\Desktop\hera-cad\SNAP\components\CAPC3216X180N_C239.ipt
- C:\Users\Dave\Desktop\hera-cad\SNAP\components\CAPC3216X180N_C246.ipt
- C:\Users\Dave\Desktop\hera-cad\SNAP\components\CAPC3216X180N_C255.ipt
- C:\Users\Dave\Desktop\hera-cad\SNAP\components\CAPC3216X180N_C264.ipt
- C:\Users\Dave\Desktop\hera-cad\SNAP\components\CAPC3216X180N_C248.ipt
- C:\Users\Dave\Desktop\hera-cad\SNAP\components\CAPC3216X180N_C257.ipt
- C:\Users\Dave\Desktop\hera-cad\SNAP\components\CAPC3216X180N_C266.ipt
- C:\Users\Dave\Desktop\hera-cad\SNAP\components\CAPC3216X180N_C268.ipt
- C:\Users\Dave\Desktop\hera-cad\SNAP\components\CAPC3216X180N_C290.ipt
- C:\Users\Dave\Desktop\hera-cad\SNAP\components\CAPMP7343X310N-ALT1_C137.ipt
- C:\Users\Dave\Desktop\hera-cad\SNAP\components\CAPMP7343X310N-ALT1_C233.ipt
- C:\Users\Dave\Desktop\hera-cad\SNAP\components\CAPMP7343X310N-ALT1_C240.ipt
- C:\Users\Dave\Desktop\hera-cad\SNAP\components\CAPMP7343X310N-ALT1_C247.ipt
- C:\Users\Dave\Desktop\hera-cad\SNAP\components\CAPMP7343X310N-ALT1_C249.ipt
- C:\Users\Dave\Desktop\hera-cad\SNAP\components\CAPMP7343X310N-ALT1_C256.ipt
- C:\Users\Dave\Desktop\hera-cad\SNAP\components\CAPMP7343X310N-ALT1_C258.ipt
- C:\Users\Dave\Desktop\hera-cad\SNAP\components\CAPMP7343X310N-ALT1_C265.ipt
- C:\Users\Dave\Desktop\hera-cad\SNAP\components\CAPMP7343X310N-ALT1_C267.ipt
- C:\Users\Dave\Desktop\hera-cad\SNAP\components\CAPC3225X270N_C414.ipt
- C:\Users\Dave\Desktop\hera-cad\SNAP\components\CAPC3225X270N_C142.ipt
- C:\Users\Dave\Desktop\hera-cad\SNAP\components\CAPC3225X270N_C147.ipt
- C:\Users\Dave\Desktop\hera-cad\SNAP\components\CAPC3225X270N_C198.ipt
- C:\Users\Dave\Desktop\hera-cad\SNAP\components\CAPC3225X270N_C199.ipt
- C:\Users\Dave\Desktop\hera-cad\SNAP\components\CAPC3225X270N_C200.ipt
- C:\Users\Dave\Desktop\hera-cad\SNAP\components\CAPC3225X270N_C201.ipt
- C:\Users\Dave\Desktop\hera-cad\SNAP\components\CAPC3225X270N_C202.ipt
- C:\Users\Dave\Desktop\hera-cad\SNAP\components\CAPC3225X270N_C203.ipt
- C:\Users\Dave\Desktop\hera-cad\SNAP\components\CAPC3225X270N_C204.ipt
- C:\Users\Dave\Desktop\hera-cad\SNAP\components\CAPC3225X270N_C205.ipt
- C:\Users\Dave\Desktop\hera-cad\SNAP\components\CAPC3225X270N_C208.ipt
- C:\Users\Dave\Desktop\hera-cad\SNAP\components\CAPC2012X105N_C162.ipt
- C:\Users\Dave\Desktop\hera-cad\SNAP\components\CAPC1005X50N_C170.ipt
- C:\Users\Dave\Desktop\hera-cad\SNAP\components\CAPAE830X1050D995DD305L335N_C191.ipt
- C:\Users\Dave\Desktop\hera-cad\SNAP\components\CAPAE830X1050D995DD305L335N_C230.ipt
- C:\Users\Dave\Desktop\hera-cad\SNAP\components\CAPAE830X1050D995DD305L335N_C237.ipt
- C:\Users\Dave\Desktop\hera-cad\SNAP\components\CAPAE830X1050D995DD305L335N_C244.ipt
- C:\Users\Dave\Desktop\hera-cad\SNAP\components\CAPAE830X1050D995DD305L335N_C253.ipt
- C:\Users\Dave\Desktop\hera-cad\SNAP\components\CAPAE830X1050D995DD305L335N_C262.ipt
- C:\Users\Dave\Desktop\hera-cad\SNAP\components\CAPMP7343X180N-ALT1_C402.ipt
- C:\Users\Dave\Desktop\hera-cad\SNAP\components\CAPMP7343X180N-ALT1_C413.ipt
- C:\Users\Dave\Desktop\hera-cad\SNAP\components\CAPMP7343X180N-ALT1_C400.ipt
- C:\Users\Dave\Desktop\hera-cad\SNAP\components\CAPMP7343X180N-ALT1_C401.ipt
- C:\Users\Dave\Desktop\hera-cad\SNAP\components\CAPMP7343X180N-ALT1_C206.ipt
- C:\Users\Dave\Desktop\hera-cad\SNAP\components\CAPMP7343X180N-ALT1_C207.ipt
- C:\Users\Dave\Desktop\hera-cad\SNAP\components\CAPC2012X140N_C419.ipt
- C:\Users\Dave\Desktop\hera-cad\SNAP\components\CAPC2012X140N_C420.ipt
- C:\Users\Dave\Desktop\hera-cad\SNAP\components\CAPC2012X140N_C410.ipt
- C:\Users\Dave\Desktop\hera-cad\SNAP\components\CAPC2012X140N_C418.ipt
- C:\Users\Dave\Desktop\hera-cad\SNAP\components\CAPC2012X140N_C417.ipt
- C:\Users\Dave\Desktop\hera-cad\SNAP\components\CAPC2012X140N_C416.ipt
- C:\Users\Dave\Desktop\hera-cad\SNAP\components\CAPC2012X140N_C415.ipt
- C:\Users\Dave\Desktop\hera-cad\SNAP\components\CAPC2012X140N_C412.ipt
- C:\Users\Dave\Desktop\hera-cad\SNAP\components\CAPC2012X140N_C411.ipt
- C:\Users\Dave\Desktop\hera-cad\SNAP\components\CAPC2012X140N_C408.ipt
- C:\Users\Dave\Desktop\hera-cad\SNAP\components\CAPC2012X140N_C409.ipt
- C:\Users\Dave\Desktop\hera-cad\SNAP\components\CAPC2012X140N_C404.ipt
- C:\Users\Dave\Desktop\hera-cad\SNAP\components\CAPC2012X140N_C407.ipt
- C:\Users\Dave\Desktop\hera-cad\SNAP\components\CAPC2012X140N_C406.ipt
- C:\Users\Dave\Desktop\hera-cad\SNAP\components\CAPC2012X140N_C405.ipt
- C:\Users\Dave\Desktop\hera-cad\SNAP\components\CAPC2012X140N_C403.ipt
- C:\Users\Dave\Desktop\hera-cad\SNAP\components\CAPC2012X140N_C209.ipt
- C:\Users\Dave\Desktop\hera-cad\SNAP\components\CAPC2012X140N_C210.ipt
- C:\Users\Dave\Desktop\hera-cad\SNAP\components\CAPC2012X140N_C211.ipt
- C:\Users\Dave\Desktop\hera-cad\SNAP\components\CAPC2012X140N_C272.ipt
- C:\Users\Dave\Desktop\hera-cad\SNAP\components\CAPC2012X140N_C274.ipt
- C:\Users\Dave\Desktop\hera-cad\SNAP\components\CAPC2012X140N_C294.ipt
- C:\Users\Dave\Desktop\hera-cad\SNAP\components\CAPC2012X140N_C296.ipt
- C:\Users\Dave\Desktop\hera-cad\SNAP\components\CAPC2012X140N_C133.ipt
- C:\Users\Dave\Desktop\hera-cad\SNAP\components\CAPC2012X140N_C130.ipt
- C:\Users\Dave\Desktop\hera-cad\SNAP\components\CAPC2012X140N_C126.ipt
- C:\Users\Dave\Desktop\hera-cad\SNAP\components\CAPC2012X140N_C125.ipt
- C:\Users\Dave\Desktop\hera-cad\SNAP\components\CAPC2012X140N_C122.ipt
- C:\Users\Dave\Desktop\hera-cad\SNAP\components\CAPC2012X140N_C118.ipt
- C:\Users\Dave\Desktop\hera-cad\SNAP\components\CAPC0603X30L_C278.ipt
- C:\Users\Dave\Desktop\hera-cad\SNAP\components\CAPC0603X30L_C281.ipt
- C:\Users\Dave\Desktop\hera-cad\SNAP\components\CAPC0603X30L_C283.ipt
- C:\Users\Dave\Desktop\hera-cad\SNAP\components\CAPC0603X30L_C288.ipt
- C:\Users\Dave\Desktop\hera-cad\SNAP\components\CAPC0603X30L_C300.ipt
- C:\Users\Dave\Desktop\hera-cad\SNAP\components\CAPC0603X30L_C303.ipt
- C:\Users\Dave\Desktop\hera-cad\SNAP\components\CAPC0603X30L_C305.ipt
- C:\Users\Dave\Desktop\hera-cad\SNAP\components\CAPC0603X30L_C310.ipt
- C:\Users\Dave\Desktop\hera-cad\SNAP\components\SOD3717X135_D10.ipt
- C:\Users\Dave\Desktop\hera-cad\SNAP\components\SOD3717X135_D9.ipt
- C:\Users\Dave\Desktop\hera-cad\SNAP\components\LEDM180X60X60N_DS1.ipt
- C:\Users\Dave\Desktop\hera-cad\SNAP\components\LEDM180X60X60N_DS10.ipt
- C:\Users\Dave\Desktop\hera-cad\SNAP\components\LEDM180X60X60N_DS11.ipt
- C:\Users\Dave\Desktop\hera-cad\SNAP\components\LEDM180X60X60N_DS4.ipt
- C:\Users\Dave\Desktop\hera-cad\SNAP\components\LEDM180X60X60N_DS5.ipt
- C:\Users\Dave\Desktop\hera-cad\SNAP\components\LEDM180X60X60N_DS7.ipt
- C:\Users\Dave\Desktop\hera-cad\SNAP\components\LEDM180X60X60N_DS8.ipt
- C:\Users\Dave\Desktop\hera-cad\SNAP\components\LEDM180X60X60N_DS9.ipt
- C:\Users\Dave\Desktop\hera-cad\SNAP\components\LEDM180X60X60N_DS2.ipt
- C:\Users\Dave\Desktop\hera-cad\SNAP\components\LEDM180X60X60N_DS3.ipt
- C:\Users\Dave\Desktop\hera-cad\SNAP\components\INDM4532X340N_L1.ipt
- C:\Users\Dave\Desktop\hera-cad\SNAP\components\INDM4532X340N_L10.ipt
- C:\Users\Dave\Desktop\hera-cad\SNAP\components\INDM4532X340N_L11.ipt
- C:\Users\Dave\Desktop\hera-cad\SNAP\components\INDM4532X340N_L12.ipt
- C:\Users\Dave\Desktop\hera-cad\SNAP\components\INDM4532X340N_L2.ipt
- C:\Users\Dave\Desktop\hera-cad\SNAP\components\INDM4532X340N_L3.ipt
- C:\Users\Dave\Desktop\hera-cad\SNAP\components\INDM4532X340N_L4.ipt
- C:\Users\Dave\Desktop\hera-cad\SNAP\components\INDM4532X340N_L5.ipt
- C:\Users\Dave\Desktop\hera-cad\SNAP\components\INDM4532X340N_L6.ipt
- C:\Users\Dave\Desktop\hera-cad\SNAP\components\INDM4532X340N_L8.ipt
- C:\Users\Dave\Desktop\hera-cad\SNAP\components\INDM4532X340N_L7.ipt
- C:\Users\Dave\Desktop\hera-cad\SNAP\components\INDM4532X340N_L9.ipt
- C:\Users\Dave\Desktop\hera-cad\SNAP\components\INDC2012X110N_L14.ipt
- C:\Users\Dave\Desktop\hera-cad\SNAP\components\INDC2012X110N_L13.ipt
- C:\Users\Dave\Desktop\hera-cad\SNAP\components\INDM9630X305N_L15.ipt
- C:\Users\Dave\Desktop\hera-cad\SNAP\components\INDM9630X305N_L16.ipt
- C:\Users\Dave\Desktop\hera-cad\SNAP\components\INDM9630X305N_L17.ipt
- C:\Users\Dave\Desktop\hera-cad\SNAP\components\INDM9630X305N_L18.ipt
- C:\Users\Dave\Desktop\hera-cad\SNAP\components\INDM9630X305N_L19.ipt
- C:\Users\Dave\Desktop\hera-cad\SNAP\components\INDC1608X95L-ALT1_L20.ipt
- C:\Users\Dave\Desktop\hera-cad\SNAP\components\INDC1608X95L-ALT1_L21.ipt
- C:\Users\Dave\Desktop\hera-cad\SNAP\components\INDC1608X95L-ALT1_L23.ipt
- C:\Users\Dave\Desktop\hera-cad\SNAP\components\INDC1608X95L-ALT1_L22.ipt